# Autodesk Inventor assembly: PCB completa
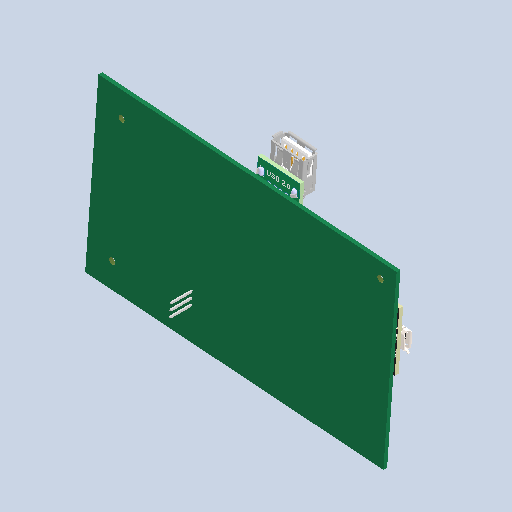
[picture p0: Inventor's stored thumbnail of the model, 512x512]
Saved by Autodesk Inventor 2023 (Build 270158000, 158)
## iProperties
Created: 2022-12-30
Part Number: PCB completa
Document SubType Name: Assembly
Designer: Gabriele
Author: Gabriele
## Documents named in this file (7)
- C:\Users\Gabriele\Desktop\Progetto Lab\AY2223_I_Project-2\3D\Case\PCB completa.iam
- C:\Users\Gabriele\Desktop\Progetto Lab\AY2223_I_Project-2\3D\Case\PCB.ipt
- C:\Users\Gabriele\Desktop\Progetto Lab\AY2223_I_Project-2\3D\Case\PROTOTYPING KIT - PSoC 5LP.ipt
- C:\Users\Gabriele\Desktop\Progetto Lab\AY2223_I_Project-2\3D\Case\Board connector.ipt
- C:\Users\Gabriele\Desktop\Progetto Lab\AY2223_I_Project-2\3D\Case\USB2A_Female_DIP2,54_PCB_adapter board.ipt
- C:\Users\Gabriele\Desktop\Progetto Lab\AY2223_I_Project-2\3D\Case\HC-05.ipt
- C:\Users\Gabriele\Desktop\Progetto Lab\AY2223_I_Project-2\3D\Case\L7805.ipt
## Components (7 placed, 6 different names)
1. PCB:1 — Coincidente:1, Allineato:1, Allineato:2, Coincidente:2, Coincidente:4, Coincidente:6, Angolo:1, Coincidente:13, Coincidente:14, Angolo:3, Coincidente:15, Allineato:7, Allineato:8, Allineato:9, Allineato:10
2. PROTOTYPING KIT - PSoC 5LP:1 — Coincidente:1, Allineato:1, Allineato:2, Coincidente:3, Allineato:3, Allineato:4
3. Board connector:1 — Coincidente:2, Coincidente:3, Allineato:3, Coincidente:5
4. Board connector:2 — Coincidente:4, Allineato:4, Coincidente:5
5. USB2A_Female_DIP2,54_PCB_adapter board:1 — Coincidente:6, Angolo:1, Allineato:9, Allineato:10
6. HC-05:1 — Coincidente:13, Coincidente:14, Angolo:3
7. L7805:1 — Coincidente:15, Allineato:7, Allineato:8
## Relationships (19: Mate 9, Flush 8, Angle 2)
- Coincidente:1 [Mate] (6 mm): PCB:1 ↔ PROTOTYPING KIT - PSoC 5LP:1
- Allineato:1 [Flush] (20 mm): PCB:1 ↔ PROTOTYPING KIT - PSoC 5LP:1
- Allineato:2 [Flush] (5 mm): PCB:1 ↔ PROTOTYPING KIT - PSoC 5LP:1
- Coincidente:2 [Mate]: PCB:1 ↔ Board connector:1
- Coincidente:3 [Mate] (1 mm): PROTOTYPING KIT - PSoC 5LP:1 ↔ Board connector:1
- Allineato:3 [Flush] (0.4 mm): PROTOTYPING KIT - PSoC 5LP:1 ↔ Board connector:1
- Coincidente:4 [Mate]: PCB:1 ↔ Board connector:2
- Allineato:4 [Flush] (1 mm): PROTOTYPING KIT - PSoC 5LP:1 ↔ Board connector:2
- Coincidente:5 [Mate] (17.4 mm): Board connector:1 ↔ Board connector:2
- Coincidente:6 [Mate] (3 mm): PCB:1 ↔ USB2A_Female_DIP2,54_PCB_adapter board:1
- Angolo:1 [Angle] (0 deg): PCB:1 ↔ USB2A_Female_DIP2,54_PCB_adapter board:1
- Coincidente:13 [Mate]: PCB:1 ↔ HC-05:1
- Coincidente:14 [Mate] (-44 mm): PCB:1 ↔ HC-05:1
- Angolo:3 [Angle] (0 deg): PCB:1 ↔ HC-05:1
- Coincidente:15 [Mate] (-10 mm): PCB:1 ↔ L7805:1
- Allineato:7 [Flush] (12 mm): PCB:1 ↔ L7805:1
- Allineato:8 [Flush] (41 mm): PCB:1 ↔ L7805:1
- Allineato:9 [Flush] (45.1 mm): PCB:1 ↔ USB2A_Female_DIP2,54_PCB_adapter board:1
- Allineato:10 [Flush] (-3.5 mm): PCB:1 ↔ USB2A_Female_DIP2,54_PCB_adapter board:1
